# Autodesk Inventor assembly: ensamble_general
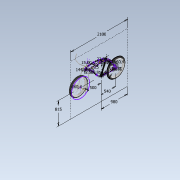
[picture p0: Inventor's stored thumbnail of the model, 180x180]
Saved by Autodesk Inventor 2021 (Build 250183000, 183)
## iProperties
Created: 2021-04-10
Part Number: ensamble_general
Document SubType Name: Assembly
Designer: j2seb
Author: j2seb
## Documents named in this file (4)
- C:\Git\Proyecto_APM\02 Inventor\ensamble_general.iam
- C:\Git\Proyecto_APM\02 Inventor\Marco_Bicicleta.iam
- C:\Git\Proyecto_APM\02 Inventor\Manubrio.ipt
- C:\Git\Proyecto_APM\02 Inventor\Ensamble_Llanta.iam
## Components (4 placed, 3 different names)
1. Marco_Bicicleta:1 [sub-assembly] — Coincidencia:1, Coincidencia:2, Coincidencia:3
2. Manubrio:1 — Coincidencia:1
3. Ensamble_Llanta:1 [sub-assembly] — Coincidencia:2
4. Ensamble_Llanta:2 [sub-assembly] — Coincidencia:4
## Relationships (5: Mate 4, Angle 1)
- Coincidencia:1 [Mate]: Marco_Bicicleta:1 ↔ Manubrio:1
- Coincidencia:2 [Mate]: Marco_Bicicleta:1 ↔ Ensamble_Llanta:1
- Coincidencia:3 [Mate]: Marco_Bicicleta:1
- Ángulo:1 [Angle] (0 deg)
- Coincidencia:4 [Mate]: Ensamble_Llanta:2
